# Autodesk Inventor assembly: door_w_glass
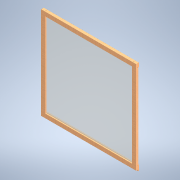
[picture p0: Inventor's stored thumbnail of the model, 180x180]
Saved by Autodesk Inventor 2020 (Build 240168000, 168)
## iProperties
Created: 2020-05-19
Part Number: door_w_glass
Document SubType Name: Assembly
Designer: kolbe
Author: kolbe
## Documents named in this file (3)
- C:\Users\kolbe\Documents\GitHub\Terrarium\door\door_w_glass.iam
- C:\Users\kolbe\Documents\GitHub\Terrarium\door\door_wo_glass.iam
- C:\Users\kolbe\Documents\GitHub\Terrarium\door\door glass.ipt
## Components (2 placed, 2 different names)
1. door_wo_glass:1 [sub-assembly] — Mate:1, Mate:2
2. door glass:1 — Mate:1, Mate:2
## Relationships (2: Mate 2)
- Mate:1: door_wo_glass:1 ↔ door glass:1
- Mate:2: door_wo_glass:1 ↔ door glass:1
